# Autodesk Inventor assembly: Stepper Motor
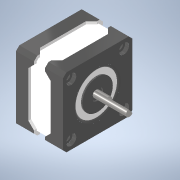
[picture p0: Inventor's stored thumbnail of the model, 180x180]
Saved by Autodesk Inventor 2021 (Build 250183000, 183)
## iProperties
Created: 2020-12-15
Part Number: Stepper Motor
Document SubType Name: Assembly
Designer: bestm
Author: bestm
## Documents named in this file (3)
- E:\Downloads\Rotary Actuator\Rotary Actuator\Stepper Motor.iam
- E:\Downloads\Rotary Actuator\Rotary Actuator\Stepper Motor Housing.ipt
- E:\Downloads\Rotary Actuator\Rotary Actuator\Stepper Motor Axle.ipt
## Components (2 placed, 2 different names)
1. Stepper Motor Housing:1 — Mate:1, Mate:2
2. Stepper Motor Axle:1 — Mate:1, Mate:2
## Relationships (2: Mate 2)
- Mate:1: Stepper Motor Housing:1 ↔ Stepper Motor Axle:1
- Mate:2: Stepper Motor Housing:1 ↔ Stepper Motor Axle:1
